# Autodesk Inventor assembly: Camera with 35mm
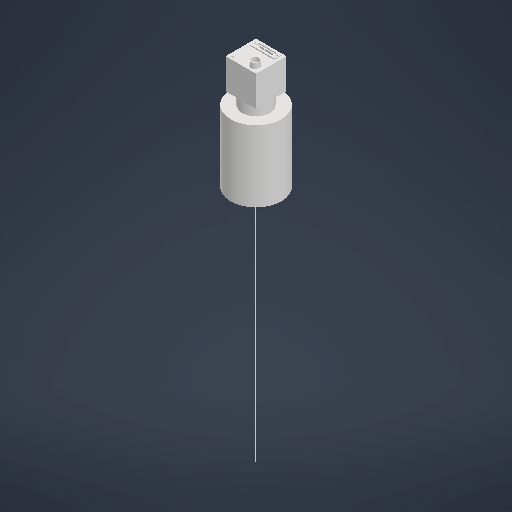
[picture p0: Inventor's stored thumbnail of the model, 512x512]
Saved by Autodesk Inventor 2026.2 (Build 302298000, 298)
## iProperties
Created: 2026-02-27
Part Number: Camera with 35mm
Document SubType Name: Assembly
Designer: mumin
Author: mumin
## Documents named in this file (3)
- C:\GitHub\In-situ-monitoring-of-powder-bed-fusion-additive-manufacturing\system_development\Mithril\v0.4\Camera with 35mm.iam
- C:\GitHub\In-situ-monitoring-of-powder-bed-fusion-additive-manufacturing\system_development\Mithril\v0.4\OpticalCamera.ipt
- C:\GitHub\In-situ-monitoring-of-powder-bed-fusion-additive-manufacturing\system_development\Mithril\v0.4\35mmLens.ipt
## Components (2 placed, 2 different names)
1. OpticalCamera:1 — Insert:1
2. 35mmLens:1 — Insert:1
## Relationships (1: Insert 1)
- Insert:1: OpticalCamera:1 ↔ 35mmLens:1
